# Autodesk Inventor assembly: motorized
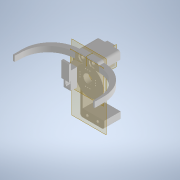
[picture p0: Inventor's stored thumbnail of the model, 180x180]
Saved by Autodesk Inventor 2020 (Build 240168000, 168)
## iProperties
Created: 2019-05-07
Part Number: motorized
Document SubType Name: Assembly
Designer: erwin
Author: erwin
## Documents named in this file (6)
- D:\GitHub\ProtoSwitchBoard\design\pin-header_cutter\new\motorized.iam
- D:\GitHub\ProtoSwitchBoard\design\pin-header_cutter\new\funnel.ipt
- D:\GitHub\ProtoSwitchBoard\design\pin-header_cutter\new\fence.ipt
- D:\GitHub\ProtoSwitchBoard\design\pin-header_cutter\new\bracket.ipt
- D:\GitHub\ProtoSwitchBoard\design\pin-header_cutter\new\leg.ipt
- D:\GitHub\ProtoSwitchBoard\design\pin-header_cutter\new\blade.ipt
## Components (5 placed, 5 different names)
1. funnel:1 — Flush:1, Flush:2
2. fence:1 — Flush:1, Flush:2, Flush:3
3. bracket:1 — Flush:3, Flush:4, Flush:5
4. leg:1 — Flush:4, Flush:5, Flush:6
5. blade:1 — Flush:6
## Relationships (6: Flush 6)
- Flush:1: funnel:1 ↔ fence:1
- Flush:2: funnel:1 ↔ fence:1
- Flush:3: fence:1 ↔ bracket:1
- Flush:4: bracket:1 ↔ leg:1
- Flush:5: bracket:1 ↔ leg:1
- Flush:6: leg:1 ↔ blade:1
